# Autodesk Inventor assembly: eto
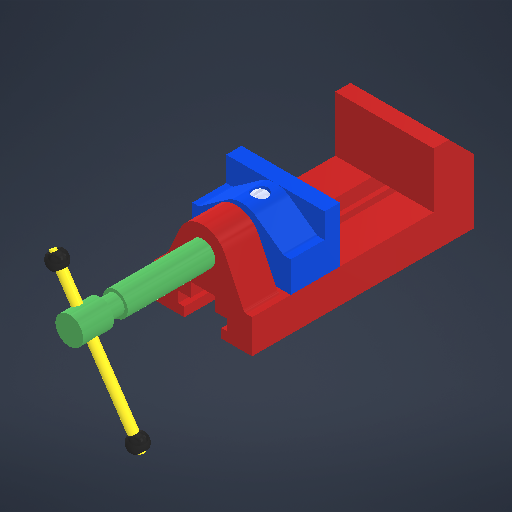
[picture p0: Inventor's stored thumbnail of the model, 512x512]
Saved by Autodesk Inventor 2025.4 (Build 294407000, 407)
## iProperties
Created: 2021-11-18
Part Number: eto
Description: STEP AP214
Document SubType Name: Assembly
Designer: VuQuan
Sending System: SolidWorks 2020
Preprocessor: SwSTEP 2.0
Title: eto.STEP
Revision Number: ANY
## Documents named in this file (9)
- D:\Edu\4CHaUI-Inventor\Assambly\B1\eto\eto.iam
- D:\Edu\4CHaUI-Inventor\Assambly\B1\eto\Bar Globes.ipt
- D:\Edu\4CHaUI-Inventor\Assambly\B1\eto\Base.ipt
- D:\Edu\4CHaUI-Inventor\Assambly\B1\eto\Base Plate.ipt
- D:\Edu\4CHaUI-Inventor\Assambly\B1\eto\Clamping Plate.ipt
- D:\Edu\4CHaUI-Inventor\Assambly\B1\eto\jaw screw.ipt
- D:\Edu\4CHaUI-Inventor\Assambly\B1\eto\Oval Fillister.ipt
- D:\Edu\4CHaUI-Inventor\Assambly\B1\eto\truc.ipt
- D:\Edu\4CHaUI-Inventor\Assambly\B1\eto\VICE.ipt
## Components (10 placed, 10 different names)
1. Bar Globes_1 — Mate:9, Mate:10, Tangent:1
2. Base_2 — Mate:4, Flush:1, Mate:6, Mate:7, Mate:13, Insert:3, Insert:4, Insert:5, Insert:6
3. Base Plate_3 — Insert:3, Insert:4
4. Clamping Plate_4 — Insert:7, Insert:8
5. jaw screw_5 — Mate:3, Insert:1, Tangent:1
6. Oval Fillister_6 — Insert:2
7. truc_7 — Mate:3, Mate:9, Mate:10, Mate:11, Mate:12
8. VICE_8 — Mate:6, Mate:7, Mate:13, Insert:1, Insert:2, Insert:7, Insert:8
9. Bar Globes_9 — Mate:11, Mate:12
10. Base Plate_10 — Insert:5, Insert:6
## Relationships (19: Mate 9, Insert 8, Flush 1, Tangent 1)
- Mate:3: jaw screw_5 ↔ truc_7
- Mate:4: Base_2
- Flush:1: Base_2
- Mate:6: Base_2 ↔ VICE_8
- Mate:7: Base_2 ↔ VICE_8
- Mate:9: Bar Globes_1 ↔ truc_7
- Mate:10: Bar Globes_1 ↔ truc_7
- Mate:11: truc_7 ↔ Bar Globes_9
- Mate:12: truc_7 ↔ Bar Globes_9
- Mate:13: Base_2 ↔ VICE_8
- Insert:1: jaw screw_5 ↔ VICE_8
- Insert:2: Oval Fillister_6 ↔ VICE_8
- Insert:3: Base_2 ↔ Base Plate_3
- Insert:4: Base_2 ↔ Base Plate_3
- Insert:5: Base_2 ↔ Base Plate_10
- Insert:6: Base_2 ↔ Base Plate_10
- Insert:7: Clamping Plate_4 ↔ VICE_8
- Insert:8: Clamping Plate_4 ↔ VICE_8
- Tangent:1: Bar Globes_1 ↔ jaw screw_5
